# Autodesk Inventor assembly: robot with small motors
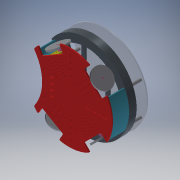
[picture p0: Inventor's stored thumbnail of the model, 180x180]
Saved by Autodesk Inventor 2016 (Build 200138000, 138)
## iProperties
Created: 2015-08-21
Part Number: robot with small motors
Document SubType Name: Assembly
Designer: TFHulbert
Author: TFHulbert
## Documents named in this file (11)
- D:\Dropbox\SHF Robotics\design\robot with small motors.iam
- D:\Dropbox\SHF Robotics\design\Bottom Plate.ipt
- D:\Dropbox\SHF Robotics\design\Goal.ipt
- D:\Dropbox\SHF Robotics\design\TSOP Plate.ipt
- D:\Dropbox\SHF Robotics\design\small spacer.ipt
- D:\Dropbox\SHF Robotics\design\Middle plate.ipt
- D:\Dropbox\SHF Robotics\design\small motor mount.ipt
- D:\Dropbox\SHF Robotics\design\small motor.ipt
- D:\Dropbox\SHF Robotics\design\wheel small.ipt
- D:\Dropbox\SHF Robotics\design\bottom pcb.ipt
- D:\Dropbox\SHF Robotics\design\back plate.ipt
## Components (22 placed, 10 different names)
1. Bottom Plate:1 — Mate:1, Mate:30, Mate:31, Mate:47, Mate:48, Mate:49, Mate:56, Mate:57, Mate:58, Mate:64, Mate:65, Mate:66, Mate:67, Mate:72, Mate:73, Mate:74, Mate:78, Mate:79, Mate:80, Mate:92, Mate:93, Mate:94, Mate:104, Mate:105, Mate:106, Mate:107, Mate:108
2. Goal:1 — Mate:1, Mate:92, Mate:93, Mate:94, Mate:95, Mate:96, Mate:97
3. TSOP Plate:1 — Mate:95, Mate:96, Mate:97, Mate:109, Mate:110, Mate:111, Mate:112, Mate:113, Mate:114, Mate:115, Mate:116, Mate:117
4. small motor mount:2 — Mate:30, Mate:31, Mate:32, Mate:33, Mate:34, Mate:56, Mate:57, Mate:58
5. small motor:1 — Mate:32, Mate:33, Mate:34, Mate:45, Mate:46
6. wheel small:1 — Mate:45, Mate:46
7. small motor:4 — Mate:50, Mate:51, Mate:52, Mate:68, Mate:69
8. small motor mount:4 — Mate:47, Mate:48, Mate:49, Mate:50, Mate:51, Mate:52
9. small motor — Mate:53, Mate:54, Mate:55, Mate:70, Mate:71, Mate:81, Mate:82, Mate:83, Mate:84, Mate:85
10. small motor mount — Mate:53, Mate:54, Mate:55, Mate:66, Mate:67, Mate:78, Mate:79, Mate:80, Mate:81, Mate:82, Mate:83
11. small motor mount:3 — Mate:59, Mate:60, Mate:61, Mate:64, Mate:65, Mate:72, Mate:73, Mate:74, Mate:75, Mate:76
12. small motor:2 — Mate:59, Mate:60, Mate:61, Mate:62, Mate:63, Mate:75, Mate:76, Mate:77
13. wheel small:4 — Mate:62, Mate:63, Mate:77
14. wheel small:2 — Mate:70, Mate:71, Mate:84, Mate:85
15. wheel small:3 — Mate:68, Mate:69
16. bottom pcb:1 — Mate:104, Mate:105, Mate:106
17. back plate:1 — Mate:107, Mate:108, Mate:109
18. small spacer:1 — Mate:116, Mate:117, Mate:119
19. small spacer:2 — Mate:114, Mate:115, Mate:118
20. small spacer:3 — Mate:112, Mate:113
21. small spacer:4 — Mate:110, Mate:111, Mate:120
22. Middle plate:1 — Mate:118, Mate:119, Mate:120
## Relationships (71: Mate 70, Flush 1)
- Mate:1: Bottom Plate:1 ↔ Goal:1
- Mate:30: Bottom Plate:1 ↔ small motor mount:2
- Mate:31: Bottom Plate:1 ↔ small motor mount:2
- Mate:32: small motor mount:2 ↔ small motor:1
- Mate:33: small motor mount:2 ↔ small motor:1
- Mate:34: small motor mount:2 ↔ small motor:1
- Mate:45: small motor:1 ↔ wheel small:1
- Mate:46: small motor:1 ↔ wheel small:1
- Flush:1
- Mate:47: Bottom Plate:1 ↔ small motor mount:4
- Mate:48: Bottom Plate:1 ↔ small motor mount:4
- Mate:49: Bottom Plate:1 ↔ small motor mount:4
- Mate:50: small motor:4 ↔ small motor mount:4
- Mate:51: small motor:4 ↔ small motor mount:4
- Mate:52: small motor:4 ↔ small motor mount:4
- Mate:53: small motor ↔ small motor mount
- Mate:54: small motor ↔ small motor mount
- Mate:55: small motor ↔ small motor mount
- Mate:56: Bottom Plate:1 ↔ small motor mount:2
- Mate:57: Bottom Plate:1 ↔ small motor mount:2
- Mate:58: Bottom Plate:1 ↔ small motor mount:2
- Mate:59: small motor mount:3 ↔ small motor:2
- Mate:60: small motor mount:3 ↔ small motor:2
- Mate:61: small motor mount:3 ↔ small motor:2
- Mate:62: small motor:2 ↔ wheel small:4
- Mate:63: small motor:2 ↔ wheel small:4
- Mate:64: Bottom Plate:1 ↔ small motor mount:3
- Mate:65: Bottom Plate:1 ↔ small motor mount:3
- Mate:66: Bottom Plate:1 ↔ small motor mount
- Mate:67: Bottom Plate:1 ↔ small motor mount
- Mate:68: small motor:4 ↔ wheel small:3
- Mate:69: small motor:4 ↔ wheel small:3
- Mate:70: small motor ↔ wheel small:2
- Mate:71: small motor ↔ wheel small:2
- Mate:72: Bottom Plate:1 ↔ small motor mount:3
- Mate:73: Bottom Plate:1 ↔ small motor mount:3
- Mate:74: Bottom Plate:1 ↔ small motor mount:3
- Mate:75: small motor mount:3 ↔ small motor:2
- Mate:76: small motor mount:3 ↔ small motor:2
- Mate:77: small motor:2 ↔ wheel small:4
- Mate:78: Bottom Plate:1 ↔ small motor mount
- Mate:79: Bottom Plate:1 ↔ small motor mount
- Mate:80: Bottom Plate:1 ↔ small motor mount
- Mate:81: small motor ↔ small motor mount
- Mate:82: small motor ↔ small motor mount
- Mate:83: small motor ↔ small motor mount
- Mate:84: small motor ↔ wheel small:2
- Mate:85: small motor ↔ wheel small:2
- Mate:92: Bottom Plate:1 ↔ Goal:1
- Mate:93: Bottom Plate:1 ↔ Goal:1
- Mate:94: Bottom Plate:1 ↔ Goal:1
- Mate:95: Goal:1 ↔ TSOP Plate:1
- Mate:96: Goal:1 ↔ TSOP Plate:1
- Mate:97: Goal:1 ↔ TSOP Plate:1
- Mate:104: Bottom Plate:1 ↔ bottom pcb:1
- Mate:105: Bottom Plate:1 ↔ bottom pcb:1
- Mate:106: Bottom Plate:1 ↔ bottom pcb:1
- Mate:107: Bottom Plate:1 ↔ back plate:1
- Mate:108: Bottom Plate:1 ↔ back plate:1
- Mate:109: TSOP Plate:1 ↔ back plate:1
- Mate:110: TSOP Plate:1 ↔ small spacer:4
- Mate:111: TSOP Plate:1 ↔ small spacer:4
- Mate:112: TSOP Plate:1 ↔ small spacer:3
- Mate:113: TSOP Plate:1 ↔ small spacer:3
- Mate:114: TSOP Plate:1 ↔ small spacer:2
- Mate:115: TSOP Plate:1 ↔ small spacer:2
- Mate:116: TSOP Plate:1 ↔ small spacer:1
- Mate:117: TSOP Plate:1 ↔ small spacer:1
- Mate:118: small spacer:2 ↔ Middle plate:1
- Mate:119: small spacer:1 ↔ Middle plate:1
- Mate:120: small spacer:4 ↔ Middle plate:1
